# Autodesk Inventor assembly: RobotInforme1
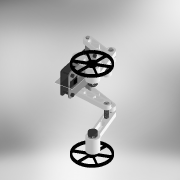
[picture p0: Inventor's stored thumbnail of the model, 180x180]
Saved by Autodesk Inventor 2021 (Build 250183000, 183)
## iProperties
Created: 2024-05-04
Part Number: RobotInforme1
Document SubType Name: Assembly
Designer: Martin
Author: Martin
## Documents named in this file (18)
- C:\Users\ASUS\OneDrive - Universidad de Antioquia\2024-1\Robótica\Proyecto\CAD\op1\RobotInforme1.iam
- C:\Users\ASUS\OneDrive - Universidad de Antioquia\2024-1\Robótica\Proyecto\CAD\37d-gearmotor-19-30-encoder.ipt
- C:\Users\ASUS\OneDrive - Universidad de Antioquia\2024-1\Robótica\Proyecto\CAD\Resorte.ipt
- C:\Users\ASUS\OneDrive - Universidad de Antioquia\2024-1\Robótica\Proyecto\CAD\op1\EslabonCodoTrasero.ipt
- C:\Users\ASUS\OneDrive - Universidad de Antioquia\2024-1\Robótica\Proyecto\CAD\op1\EslabonRodillaCadera.ipt
- C:\Users\ASUS\OneDrive - Universidad de Antioquia\2024-1\Robótica\Proyecto\CAD\op1\EslabonRuedaRodilla.ipt
- C:\Users\ASUS\OneDrive - Universidad de Antioquia\2024-1\Robótica\Proyecto\CAD\op1\Llana.ipt
- C:\Users\ASUS\Documents\Inventor\Content Center Files\R2021\en-US\BS 290 SKF(30)\BS 290 SKF - SKF 608.ipt
- C:\Users\ASUS\Documents\Inventor\Content Center Files\R2021\en-US\AS 1110\AS 1110 - M8 x 80.ipt
- C:\Users\ASUS\OneDrive - Universidad de Antioquia\2024-1\Robótica\Proyecto\CAD\op1\BaseEnsamble.iam
- C:\Users\ASUS\Documents\Inventor\Content Center Files\R2021\en-US\AS 1110\AS 1110 - M8 x 55.ipt
- C:\Users\ASUS\Documents\Inventor\Content Center Files\R2021\en-US\AS 1111\AS 1111 - M8 x 90.ipt
- C:\Users\ASUS\OneDrive - Universidad de Antioquia\2024-1\Robótica\Proyecto\CAD\37d-gearmotor-19-30-encoder_MIR4.ipt
- C:\Users\ASUS\OneDrive - Universidad de Antioquia\2024-1\Robótica\Proyecto\CAD\Resorte_MIR5.ipt
- C:\Users\ASUS\OneDrive - Universidad de Antioquia\2024-1\Robótica\Proyecto\CAD\op1\EslabonCodoTrasero_MIR4.ipt
- C:\Users\ASUS\OneDrive - Universidad de Antioquia\2024-1\Robótica\Proyecto\CAD\op1\EslabonRodillaCadera_MIR4.ipt
- C:\Users\ASUS\OneDrive - Universidad de Antioquia\2024-1\Robótica\Proyecto\CAD\op1\EslabonRuedaRodilla_MIR4.ipt
- C:\Users\ASUS\OneDrive - Universidad de Antioquia\2024-1\Robótica\Proyecto\CAD\op1\Llana_MIR2.ipt
## Components (25 placed, 17 different names)
1. 37d-gearmotor-19-30-encoder:1 — Mate:1, Mate:2, Mate:3, Mate:4
2. Resorte:1 — Mate:6, Mate:9
3. EslabonCodoTrasero:1 — Mate:7, Mate:8, Mate:21, Mate:22, Mate:26
4. EslabonRodillaCadera:1 — Mate:9, Mate:10, Mate:18, Mate:19, Mate:20
5. EslabonRuedaRodilla:1 — Mate:1, Mate:2, Mate:3, Mate:5, Mate:6, Mate:7, Mate:8, Mate:10, Mate:11, Mate:12, Mate:13, Mate:14, Mate:15, Mate:16, Mate:17, Mate:23, Mate:24
6. Llana:1 — Mate:4, Mate:5
7. BS 290 SKF 608:1 — Mate:11, Mate:12, Mate:13
8. BS 290 SKF 608:2 — Mate:14, Mate:15
9. AS 1110 - Metric M8 x 80:1 — Mate:16, Mate:17
10. BS 290 SKF 608:3 — Mate:18, Mate:19
11. BaseEnsamble:1 [sub-assembly] — Mate:20, Mate:21, Mate:22, Mate:25
12. AS 1110 - Metric M8 x 55:1 — Mate:23, Mate:24
13. AS 1111 - Metric M8 x 90:1 — Mate:25, Mate:26
14. 37d-gearmotor-19-30-encoder_MIR4:1 — Mate:32, Mate:33, Mate:34, Mate:36
15. Resorte_MIR5:1 — Mate:27, Mate:31
16. EslabonCodoTrasero_MIR4:1 — Mate:29, Mate:30, Mate:48
17. EslabonRodillaCadera_MIR4:1 — Mate:27, Mate:28, Mate:44, Mate:45
18. EslabonRuedaRodilla_MIR4:1 — Mate:28, Mate:29, Mate:30, Mate:31, Mate:32, Mate:33, Mate:34, Mate:35, Mate:37, Mate:38, Mate:39, Mate:40, Mate:41, Mate:42, Mate:43, Mate:46, Mate:47
19. Llana_MIR2:1 — Mate:35, Mate:36
20. BS 290 SKF 608:4 — Mate:37, Mate:38, Mate:39
21. BS 290 SKF 608:5 — Mate:40, Mate:41
22. AS 1110 - Metric M8 x 80:2 — Mate:42, Mate:43
23. BS 290 SKF 608:6 — Mate:44, Mate:45
24. AS 1110 - Metric M8 x 55:2 — Mate:46, Mate:47
25. AS 1111 - Metric M8 x 90:2 — Mate:48
## Relationships (48: Mate 48)
- Mate:1: 37d-gearmotor-19-30-encoder:1 ↔ EslabonRuedaRodilla:1
- Mate:2: 37d-gearmotor-19-30-encoder:1 ↔ EslabonRuedaRodilla:1
- Mate:3: 37d-gearmotor-19-30-encoder:1 ↔ EslabonRuedaRodilla:1
- Mate:4: 37d-gearmotor-19-30-encoder:1 ↔ Llana:1
- Mate:5 (5 mm): EslabonRuedaRodilla:1 ↔ Llana:1
- Mate:6: Resorte:1 ↔ EslabonRuedaRodilla:1
- Mate:7: EslabonCodoTrasero:1 ↔ EslabonRuedaRodilla:1
- Mate:8 (6.7 mm): EslabonCodoTrasero:1 ↔ EslabonRuedaRodilla:1
- Mate:9: Resorte:1 ↔ EslabonRodillaCadera:1
- Mate:10 (40 mm): EslabonRodillaCadera:1 ↔ EslabonRuedaRodilla:1
- Mate:11: EslabonRuedaRodilla:1 ↔ BS 290 SKF 608:1
- Mate:12: EslabonRuedaRodilla:1 ↔ BS 290 SKF 608:1
- Mate:13: EslabonRuedaRodilla:1 ↔ BS 290 SKF 608:1
- Mate:14: EslabonRuedaRodilla:1 ↔ BS 290 SKF 608:2
- Mate:15: EslabonRuedaRodilla:1 ↔ BS 290 SKF 608:2
- Mate:16: EslabonRuedaRodilla:1 ↔ AS 1110 - Metric M8 x 80:1
- Mate:17: EslabonRuedaRodilla:1 ↔ AS 1110 - Metric M8 x 80:1
- Mate:18: EslabonRodillaCadera:1 ↔ BS 290 SKF 608:3
- Mate:19: EslabonRodillaCadera:1 ↔ BS 290 SKF 608:3
- Mate:20: EslabonRodillaCadera:1 ↔ BaseEnsamble:1
- Mate:21: EslabonCodoTrasero:1 ↔ BaseEnsamble:1
- Mate:22: EslabonCodoTrasero:1 ↔ BaseEnsamble:1
- Mate:23: EslabonRuedaRodilla:1 ↔ AS 1110 - Metric M8 x 55:1
- Mate:24: EslabonRuedaRodilla:1 ↔ AS 1110 - Metric M8 x 55:1
- Mate:25: BaseEnsamble:1 ↔ AS 1111 - Metric M8 x 90:1
- Mate:26: EslabonCodoTrasero:1 ↔ AS 1111 - Metric M8 x 90:1
- Mate:27: Resorte_MIR5:1 ↔ EslabonRodillaCadera_MIR4:1
- Mate:28 (40 mm): EslabonRodillaCadera_MIR4:1 ↔ EslabonRuedaRodilla_MIR4:1
- Mate:29 (6.7 mm): EslabonCodoTrasero_MIR4:1 ↔ EslabonRuedaRodilla_MIR4:1
- Mate:30: EslabonCodoTrasero_MIR4:1 ↔ EslabonRuedaRodilla_MIR4:1
- Mate:31: Resorte_MIR5:1 ↔ EslabonRuedaRodilla_MIR4:1
- Mate:32: 37d-gearmotor-19-30-encoder_MIR4:1 ↔ EslabonRuedaRodilla_MIR4:1
- Mate:33: 37d-gearmotor-19-30-encoder_MIR4:1 ↔ EslabonRuedaRodilla_MIR4:1
- Mate:34: 37d-gearmotor-19-30-encoder_MIR4:1 ↔ EslabonRuedaRodilla_MIR4:1
- Mate:35 (5 mm): EslabonRuedaRodilla_MIR4:1 ↔ Llana_MIR2:1
- Mate:36: 37d-gearmotor-19-30-encoder_MIR4:1 ↔ Llana_MIR2:1
- Mate:37: EslabonRuedaRodilla_MIR4:1 ↔ BS 290 SKF 608:4
- Mate:38: EslabonRuedaRodilla_MIR4:1 ↔ BS 290 SKF 608:4
- Mate:39: EslabonRuedaRodilla_MIR4:1 ↔ BS 290 SKF 608:4
- Mate:40: EslabonRuedaRodilla_MIR4:1 ↔ BS 290 SKF 608:5
- Mate:41: EslabonRuedaRodilla_MIR4:1 ↔ BS 290 SKF 608:5
- Mate:42: EslabonRuedaRodilla_MIR4:1 ↔ AS 1110 - Metric M8 x 80:2
- Mate:43: EslabonRuedaRodilla_MIR4:1 ↔ AS 1110 - Metric M8 x 80:2
- Mate:44: EslabonRodillaCadera_MIR4:1 ↔ BS 290 SKF 608:6
- Mate:45: EslabonRodillaCadera_MIR4:1 ↔ BS 290 SKF 608:6
- Mate:46: EslabonRuedaRodilla_MIR4:1 ↔ AS 1110 - Metric M8 x 55:2
- Mate:47: EslabonRuedaRodilla_MIR4:1 ↔ AS 1110 - Metric M8 x 55:2
- Mate:48: EslabonCodoTrasero_MIR4:1 ↔ AS 1111 - Metric M8 x 90:2
